# Autodesk Inventor assembly: 上層部v2
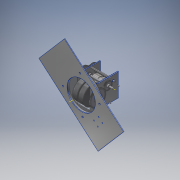
[picture p0: Inventor's stored thumbnail of the model, 180x180]
Saved by Autodesk Inventor 2019 (Build 230136000, 136)
## iProperties
Created: 2020-10-22
Part Number: 上層部v2
Material: 一般
Document SubType Name: Assembly
Designer: zhept
Author: zhept
## iProperties of the stored document _SCS  0808CP3-part.ipt
Created: 2020-09-25
Part Number: _SCS  0808CP3-part
Material: 一般
Document SubType Name: Modeling
Designer: zhept
Density: 1 g/cm^3
Appearance: 既定
Mass: 2.79624 g
Surface Area: 21.3056 cm^2
Volume: 2.79624 cm^3
Author: zhept
Revision Number: NONE
## iProperties of the stored document SC0607CB1.iam
Company: CADENAS
Created: 2020-10-25
Part Number: SC0607CB1
Material: 一般
Description: STEP AP203
Document SubType Name: Assembly
Designer: zhept
Mass: 0.54499 g
Surface Area: 6.22376 cm^2
Volume: 0.54499 cm^3
Density: 1 g/cm^3
Sending System: PARTsolutions
Title: p:/temp/worker_1/temp/exporttempdir_432_4_ZayYd/format_0/SC0607CB1.stp
Author: License CC BY-ND 4.0
Revision Number: NONE
## iProperties of the stored document _SC  0607CB1.ipt
Created: 2020-09-25
Part Number: _SC  0607CB1
Material: 一般
Document SubType Name: Modeling
Designer: zhept
Density: 1 g/cm^3
Appearance: 既定
Mass: 0.54499 g
Surface Area: 6.22376 cm^2
Volume: 0.54499 cm^3
Author: zhept
Revision Number: NONE
## iProperties of the stored document SC0809CB1.iam
Company: CADENAS
Created: 2020-10-25
Part Number: SC0809CB1
Material: 一般
Description: STEP AP203
Document SubType Name: Assembly
Designer: zhept
Mass: 1.4726 g
Surface Area: 11.5757 cm^2
Volume: 1.4726 cm^3
Density: 1 g/cm^3
Sending System: PARTsolutions
Title: p:/temp/worker_13/temp/exporttempdir_2696_289_8DYWm/format_0/SC0809CB1.stp
Author: License CC BY-ND 4.0
Revision Number: NONE
## iProperties of the stored document DS1-80_On.ipt
Created: 2020-10-25
Part Number: DS1-80_On
Material: 一般
Description: STEP AP203
Document SubType Name: Modeling
Designer: zhept
Density: 1 g/cm^3
Appearance: 既定
Company: CADENAS
Sending System: PARTsolutions
Title: p:/temp/worker_10/temp/exporttempdir_3100_306_irwf7/format_0/DS1-80_On.stp
Author: License CC BY-ND 4.0
Revision Number: NONE
## iProperties of the stored document DS1-40_On.ipt
Created: 2020-04-11
Part Number: DS1-40_On
Material: 一般
Description: STEP AP203
Document SubType Name: Modeling
Designer: zhept
Density: 1 g/cm^3
Appearance: 既定
Mass: 5.86363 g
Surface Area: 49.6933 cm^2
Volume: 5.86363 cm^3
Company: CADENAS
Sending System: PARTsolutions
Title: p:/temp/worker_5/temp/exporttempdir_324_303_oApUy/format_0/DS1-40_On.stp
Author: License CC BY-ND 4.0
Revision Number: NONE
## iProperties of the stored document _SC  0809CB1.ipt
Created: 2020-09-25
Part Number: _SC  0809CB1
Material: 一般
Document SubType Name: Modeling
Designer: zhept
Density: 1 g/cm^3
Appearance: 既定
Mass: 1.4726 g
Surface Area: 11.5757 cm^2
Volume: 1.4726 cm^3
Author: zhept
Revision Number: NONE
## iProperties of the stored document SCS0808CP3.iam
Company: CADENAS
Created: 2020-10-25
Part Number: SCS0808CP3
Material: 一般
Description: STEP AP203
Document SubType Name: Assembly
Designer: zhept
Sending System: PARTsolutions
Title: p:/temp/worker_8/temp/exporttempdir_1868_723_K7orS/format_0/SCS0808CP3.stp
Author: License CC BY-ND 4.0
Revision Number: NONE
## iProperties of the stored document DS1-50_On.ipt
Created: 2020-10-25
Part Number: DS1-50_On
Material: 一般
Description: STEP AP203
Document SubType Name: Modeling
Designer: zhept
Density: 1 g/cm^3
Appearance: 既定
Mass: 8.85233 g
Surface Area: 69.8882 cm^2
Volume: 8.85233 cm^3
Company: CADENAS
Sending System: PARTsolutions
Title: p:/temp/worker_1/temp/exporttempdir_432_85_1kcEd/format_0/DS1-50_On.stp
Author: License CC BY-ND 4.0
Revision Number: NONE
## Documents named in this file (39)
- **C:\Users\zhept\OneDrive\大学\rrst\足回り2020\上層部v2\上層部v2.iam*LocalDocs*xHo0cebq5Klpeubcj2zggdrxcOf*_SCS  0808CP3-part.ipt
- **C:\Users\zhept\OneDrive\大学\rrst\足回り2020\上層部v2\上層部v2.iam*LocalDocs*x5yppecwfCjhbezs5X0x0yqco3c*SC0607CB1.iam
- **C:\Users\zhept\OneDrive\大学\rrst\足回り2020\上層部v2\上層部v2.iam*LocalDocs*x3u5wxtziD5i0egcnFyauy2pb1f*_SC  0607CB1.ipt
- **C:\Users\zhept\OneDrive\大学\rrst\足回り2020\上層部v2\上層部v2.iam*LocalDocs*xB1pz54zd224huewxSlfgugthSh*SC0809CB1.iam
- **C:\Users\zhept\OneDrive\大学\rrst\足回り2020\上層部v2\上層部v2.iam*LocalDocs*xRp2ashovMbncuooiG1yozjblSb*_SC  0809CB1.ipt
- **C:\Users\zhept\OneDrive\大学\rrst\足回り2020\上層部v2.iam*LocalDocs*xJn5lqbh0O5ttewoeZfopalkn3b*DS1-80_On.ipt
- **C:\Users\zhept\OneDrive\大学\rrst\足回り2020\上層部v2\上層部v2.iam*LocalDocs*xI5ndwy3aVnpju2w0L5tf3rl4Mc*DS1-40_On.ipt
- **C:\Users\zhept\OneDrive\大学\rrst\足回り2020\上層部v2.iam*LocalDocs*xKvlonthoXmytuxwuY1p3cpkqQa*SCS0808CP3.iam
- **C:\Users\zhept\OneDrive\大学\rrst\足回り2020\上層部v2.iam*LocalDocs*xHo0cebq5Klpeubcj2zggdrxcOf*_SCS  0808CP3-part.ipt
- **C:\Users\zhept\OneDrive\大学\rrst\足回り2020\上層部v2\上層部v2.iam*LocalDocs*xZy5zulvjNup4u2krAgdal5x2Ub*DS1-50_On.ipt
- C:\Users\zhept\OneDrive\大学\rrst\足回り2020\上層部v2\上層部v2.iam
- C:\Users\zhept\OneDrive\大学\rrst\足回り2020\上層部v2\板2.ipt
- C:\Users\zhept\OneDrive\大学\rrst\足回り2020\上層部v2\モータ RZ-735VA.ipt
- C:\Users\zhept\OneDrive\大学\rrst\足回り2020\上層部v2\KHK_SS0530BOn.ipt
- C:\Users\zhept\OneDrive\大学\rrst\足回り2020\上層部v2\6mmベアリング.ipt
- C:\Users\zhept\OneDrive\大学\rrst\足回り2020\上層部v2\8mmベアリング.ipt
- C:\Users\zhept\OneDrive\大学\rrst\足回り2020\上層部v2\組み合わせギア_0.5-100_SSY1_15.iam
- C:\Users\zhept\OneDrive\大学\rrst\足回り2020\上層部v2\6mm軸1.ipt
- C:\Users\zhept\OneDrive\大学\rrst\足回り2020\上層部v2\セットカラー_6mm.ipt
- C:\Users\zhept\OneDrive\大学\rrst\足回り2020\上層部v2\8mm軸_1.ipt
- **C:\Users\zhept\OneDrive\大学\rrst\足回り2020\上層部v2\上層部v2.iam*LocalDocs*xKvlonthoXmytuxwuY1p3cpkqQa*SCS0808CP3.iam
- C:\Users\zhept\OneDrive\大学\rrst\足回り2020\上層部v2\8mm軸_2.ipt
- C:\Users\zhept\OneDrive\大学\rrst\足回り2020\上層部v2\HAMMER_CASTER_425ER100.ipt
- C:\Users\zhept\OneDrive\大学\rrst\足回り2020\上層部v2\フランジ.iam
- C:\Users\zhept\OneDrive\大学\rrst\足回り2020\上層部v2\板4.ipt
- **C:\Users\zhept\OneDrive\大学\rrst\足回り2020\上層部v2\上層部v2.iam*LocalDocs*xJn5lqbh0O5ttewoeZfopalkn3b*DS1-80_On.ipt
- C:\Users\zhept\OneDrive\大学\rrst\足回り2020\上層部v2\六角スペーサー.ipt
- C:\Users\zhept\OneDrive\大学\rrst\足回り2020\二つ分け角柱.ipt
- C:\Users\zhept\OneDrive\大学\rrst\足回り2020\KHK_SS295J20On\KHK_SS295J20On.ipt
- C:\Users\zhept\OneDrive\大学\rrst\足回り2020\ベアリング_145mm_inside.ipt
- C:\Users\zhept\OneDrive\大学\rrst\足回り2020\ベアリング板\ベアリング板.ipt
- C:\Users\zhept\OneDrive\大学\rrst\足回り2020\足回り試作2020_v1\ベアリング 外側.ipt
- C:\Users\zhept\OneDrive\大学\rrst\足回り2020\KHK_SS220J12On\SS2-20J12_On.ipt
- C:\Users\zhept\OneDrive\大学\rrst\足回り2020\上層部v2\SC0607CB1.stp
- C:\Users\zhept\OneDrive\大学\rrst\足回り2020\上層部v2\SC0809CB1.stp
- C:\Users\zhept\OneDrive\大学\rrst\足回り2020\上層部v2\DS1-50_On.stp
- C:\Users\zhept\OneDrive\大学\rrst\足回り2020\上層部v2\SCS0808CP3.stp
- C:\Users\zhept\OneDrive\大学\rrst\足回り2020\上層部v2\DS1-40_On.stp
- C:\Users\zhept\OneDrive\大学\rrst\足回り2020\上層部v2\DS1-80_On.stp
## Components (42 placed, 26 different names)
1. 板2:1 — 挿入:1, メイト:1, 回転:7, 挿入:19, 挿入:23, 挿入:32, 挿入:33, 挿入:34, 挿入:35
2. モータ RZ-735VA:1 — 挿入:1, 挿入:2
3. KHK_SS0530BOn:1 — 挿入:2, フラッシュ:1
4. 組み合わせギア_0.5-100_SSY1_15:1 [sub-assembly] — 円柱状:1, フラッシュ:1, 挿入:3, 挿入:4, フラッシュ:2
5. 6mm軸1:1 — 円柱状:1
6. セットカラー_6mm:1 — 挿入:3
7. セットカラー_6mm:2 — 挿入:4
8. 8mm軸_1:1 — 円柱状:2, メイト:4, 円柱状:4
9. DS1-50_On:1 — 円柱状:2, フラッシュ:2, 挿入:12
10. 8mm軸_2:1 — 円柱状:3, 円柱状:5
11. HAMMER_CASTER_425ER100:1 — 挿入:9, 挿入:10
12. HAMMER_CASTER_425ER100:2 — 挿入:9, 挿入:11
13. SCS0808CP3:2 [sub-assembly] — 挿入:11, メイト:8, メイト:10
14. SCS0808CP3:3 [sub-assembly] — 挿入:10, 円柱状:3, メイト:1
15. フランジ:1 [sub-assembly] — 挿入:12
16. DS1-40_On:1 — 円柱状:4, フラッシュ:3
17. DS1-80_On:1 — フラッシュ:3, 挿入:16, メイト:9
18. フランジ:2 [sub-assembly] — 挿入:16, 円柱状:5
19. 板4:1 — メイト:8, 回転:6, 挿入:20, 挿入:25, 挿入:27, 挿入:28, 挿入:29, 挿入:30, 挿入:31, 挿入:36, 挿入:37
20. 8mmベアリング:7 — 回転:6, メイト:9
21. 8mmベアリング:8 — 回転:7, 挿入:18
22. SC0809CB1:4 [sub-assembly] — 挿入:18
23. SC0607CB1:2 [sub-assembly] — 挿入:21
24. SC0607CB1:3 [sub-assembly] — 挿入:22
25. 6mmベアリング:2 — 挿入:19, 挿入:22
26. 6mmベアリング:3 — 挿入:20, 挿入:21
27. SC0809CB1:5 [sub-assembly] — 挿入:24
28. SC0809CB1:6 [sub-assembly] — 挿入:26
29. 8mmベアリング:9 — 挿入:23, 挿入:24
30. 8mmベアリング:10 — 挿入:25, 挿入:26
31. 六角スペーサー:1 — 挿入:27
32. 六角スペーサー:2 — 挿入:28
33. 六角スペーサー:3 — 挿入:29
34. 二つ分け角柱:1 — 挿入:30, 挿入:31
35. 二つ分け角柱:3 — 挿入:36, 挿入:37, 挿入:39
36. 二つ分け角柱:5 — 挿入:34, 挿入:35, 挿入:38
37. 二つ分け角柱:6 — 挿入:32, 挿入:33
38. KHK_SS295J20On:1 — 挿入:38, 挿入:39, 挿入:40, 挿入:41, フラッシュ:4
39. ベアリング_145mm_inside:1 — 挿入:40, 挿入:41, メイト:12
40. ベアリング板:1 — 挿入:42, 挿入:43
41. ベアリング 外側:1 — 挿入:42, 挿入:43, メイト:11
42. SS2-20J12_On:1 — フラッシュ:4
## Relationships (55: Insert 35, Mate 9, CylindricalJoint 5, Flush 4, RevoluteJoint 2)
- 挿入:1 [Insert]: 板2:1 ↔ モータ RZ-735VA:1
- 挿入:2 [Insert] (0.5 mm): モータ RZ-735VA:1 ↔ KHK_SS0530BOn:1
- 円柱状:1 [CylindricalJoint]: 組み合わせギア_0.5-100_SSY1_15:1 ↔ 6mm軸1:1
- フラッシュ:1 [Flush] (2 mm): KHK_SS0530BOn:1 ↔ 組み合わせギア_0.5-100_SSY1_15:1
- 挿入:3 [Insert]: 組み合わせギア_0.5-100_SSY1_15:1 ↔ セットカラー_6mm:1
- 挿入:4 [Insert]: 組み合わせギア_0.5-100_SSY1_15:1 ↔ セットカラー_6mm:2
- 円柱状:2 [CylindricalJoint]: 8mm軸_1:1 ↔ DS1-50_On:1
- フラッシュ:2 [Flush]: 組み合わせギア_0.5-100_SSY1_15:1 ↔ DS1-50_On:1
- 挿入:9 [Insert]: HAMMER_CASTER_425ER100:1 ↔ HAMMER_CASTER_425ER100:2
- 挿入:10 [Insert]: HAMMER_CASTER_425ER100:1 ↔ SCS0808CP3:3
- 挿入:11 [Insert]: HAMMER_CASTER_425ER100:2 ↔ SCS0808CP3:2
- 円柱状:3 [CylindricalJoint]: 8mm軸_2:1 ↔ SCS0808CP3:3
- 挿入:12 [Insert] (2 mm): DS1-50_On:1 ↔ フランジ:1
- メイト:1 [Mate] (7 mm): 板2:1 ↔ SCS0808CP3:3
- メイト:4 [Mate]: 8mm軸_1:1
- メイト:5 [Mate]
- 円柱状:4 [CylindricalJoint]: 8mm軸_1:1 ↔ DS1-40_On:1
- フラッシュ:3 [Flush]: DS1-40_On:1 ↔ DS1-80_On:1
- 挿入:16 [Insert]: DS1-80_On:1 ↔ フランジ:2
- メイト:8 [Mate] (7 mm): SCS0808CP3:2 ↔ 板4:1
- 円柱状:5 [CylindricalJoint]: 8mm軸_2:1 ↔ フランジ:2
- 回転:6 [RevoluteJoint]: 板4:1 ↔ 8mmベアリング:7
- メイト:9 [Mate]: DS1-80_On:1 ↔ 8mmベアリング:7
- 回転:7 [RevoluteJoint]: 板2:1 ↔ 8mmベアリング:8
- 挿入:18 [Insert]: 8mmベアリング:8 ↔ SC0809CB1:4
- メイト:10 [Mate]: SCS0808CP3:2
- 挿入:19 [Insert]: 板2:1 ↔ 6mmベアリング:2
- 挿入:20 [Insert]: 板4:1 ↔ 6mmベアリング:3
- 挿入:21 [Insert]: SC0607CB1:2 ↔ 6mmベアリング:3
- 挿入:22 [Insert]: SC0607CB1:3 ↔ 6mmベアリング:2
- 挿入:23 [Insert]: 板2:1 ↔ 8mmベアリング:9
- 挿入:24 [Insert]: SC0809CB1:5 ↔ 8mmベアリング:9
- 挿入:25 [Insert]: 板4:1 ↔ 8mmベアリング:10
- 挿入:26 [Insert]: SC0809CB1:6 ↔ 8mmベアリング:10
- 挿入:27 [Insert]: 板4:1 ↔ 六角スペーサー:1
- 挿入:28 [Insert]: 板4:1 ↔ 六角スペーサー:2
- 挿入:29 [Insert]: 板4:1 ↔ 六角スペーサー:3
- 挿入:30 [Insert]: 板4:1 ↔ 二つ分け角柱:1
- 挿入:31 [Insert]: 板4:1 ↔ 二つ分け角柱:1
- 挿入:32 [Insert]: 板2:1 ↔ 二つ分け角柱:6
- 挿入:33 [Insert]: 板2:1 ↔ 二つ分け角柱:6
- 挿入:34 [Insert]: 板2:1 ↔ 二つ分け角柱:5
- 挿入:35 [Insert]: 板2:1 ↔ 二つ分け角柱:5
- 挿入:36 [Insert]: 板4:1 ↔ 二つ分け角柱:3
- 挿入:37 [Insert]: 板4:1 ↔ 二つ分け角柱:3
- 挿入:38 [Insert]: 二つ分け角柱:5 ↔ KHK_SS295J20On:1
- 挿入:39 [Insert]: 二つ分け角柱:3 ↔ KHK_SS295J20On:1
- 挿入:40 [Insert]: KHK_SS295J20On:1 ↔ ベアリング_145mm_inside:1
- 挿入:41 [Insert]: KHK_SS295J20On:1 ↔ ベアリング_145mm_inside:1
- 挿入:42 [Insert]: ベアリング板:1 ↔ ベアリング 外側:1
- 挿入:43 [Insert]: ベアリング板:1 ↔ ベアリング 外側:1
- メイト:11 [Mate]: ベアリング 外側:1
- メイト:12 [Mate]: ベアリング_145mm_inside:1
- メイト:13 [Mate]
- フラッシュ:4 [Flush]: KHK_SS295J20On:1 ↔ SS2-20J12_On:1
